# Autodesk Inventor assembly: 組合檔
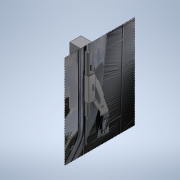
[picture p0: Inventor's stored thumbnail of the model, 180x180]
Saved by Autodesk Inventor 2020 (Build 240168000, 168)
## iProperties
Created: 2015-11-28
Part Number: 組合檔
Document SubType Name: Assembly
Designer: 設計製圖
Author: 設計製圖
## Documents named in this file (14)
- D:\資料庫\設計-3D Project\【May club 】\得利卡-車頂燈架\模型、圖面\22.01.05_設變 (未生產 )\短-車頂燈架-組合(#11.02)-總組合.iam
- D:\資料庫\設計-3D Project\材料庫\【螺絲】\止付螺絲\止付螺絲-M8-20.ipt
- D:\資料庫\設計-3D Project\【May club 】\得利卡-車頂燈架\模型、圖面\車身圖.ipt
- D:\資料庫\設計-3D Project\【May club 】\得利卡-車頂燈架\模型、圖面\得利卡-車頂導水槽.ipt
- D:\資料庫\設計-3D Project\材料庫\【螺絲】\外六角螺絲\白鐵-外六角  M6-20.ipt
- D:\資料庫\設計-3D Project\材料庫\【華司】\白鐵-平面華司-7-16-2t.ipt
- D:\資料庫\設計-3D Project\材料庫\【華司】\彈簧華司\白鐵-彈簧華司-6.ipt
- D:\資料庫\設計-3D Project\【May club 】\得利卡-車頂燈架\模型、圖面\短-車頂燈架-組合(#11.02)-生產圖面_21.11.26\製程筆記\封邊條 ( 平光黑 ) - 130L.ipt
- D:\資料庫\設計-3D Project\【May club 】\得利卡-車頂燈架\模型、圖面\短-車頂燈架-組合(#11.02)-生產圖面_21.11.26\製程筆記\背膠海綿eva 6T -  15W x 125L.ipt
- D:\資料庫\設計-3D Project\【May club 】\得利卡-車頂燈架\模型、圖面\短-車頂燈架-組合(#11.02)-生產圖面_21.11.26\製程筆記\背膠海綿eva 3T -  25W x 125L.ipt
- D:\資料庫\設計-3D Project\【May club 】\得利卡-車頂燈架\模型、圖面\短-車頂燈架-組合(#11.02)-生產圖面_21.11.26\製程筆記\背膠海綿eva 3T -  10W x 125L.ipt
- D:\資料庫\設計-3D Project\【May club 】\得利卡-車頂燈架\模型、圖面\22.01.05_設變 (未生產 )\吊架-短(R)(#01.05) - 焊接組合.iam
- D:\資料庫\設計-3D Project\【May club 】\得利卡-車頂燈架\模型、圖面\22.01.05_設變 (未生產 )\ㄇ槽(#01.05)- 焊接組合.iam
- D:\資料庫\設計-3D Project\【 鐵蹄 】\------鐵蹄工廠素材------ -\拉帽-M8.ipt
## Components (15 placed, 13 different names)
1. 吊架-短(R)(#01.05) - 焊接組合:1 [sub-assembly] — 貼合:68, 貼合:69, 齊平:13, 貼合:70, 貼合:74, 貼合:75, 齊平:15, 貼合:79, 貼合:80, 齊平:17, 貼合:81, 角度:1
2. ㄇ槽(#01.05)- 焊接組合:1 [sub-assembly] — 貼合:63, 貼合:64, 貼合:65, 貼合:66, 貼合:70, 貼合:71, 貼合:72, 貼合:73, 齊平:14, 貼合:76, 齊平:16, 齊平:17, 貼合:81, 角度:2
3. 拉帽-M8:1 — 貼合:63, 貼合:64, 貼合:67, 貼合:78
4. 拉帽-M8:2 — 貼合:65, 貼合:66, 貼合:67, 貼合:77
5. 得利卡-車頂導水槽:1
6. 車身圖:1
7. 背膠海綿eva 6T -  15W x 125L:1 — 貼合:74, 貼合:75, 齊平:15
8. 背膠海綿eva 3T -  25W x 125L:1 — 貼合:62, 貼合:72, 貼合:73, 齊平:14
9. 背膠海綿eva 3T -  10W x 125L:1 — 貼合:62, 貼合:76, 齊平:16
10. 白鐵-彈簧華司-6:1 — 貼合:49, 貼合:51, 貼合:52
11. 白鐵-平面華司-7-16-2t:1 — 貼合:48, 貼合:51, 貼合:80
12. 白鐵-外六角  M6-20:1 — 貼合:48, 貼合:49, 貼合:52, 貼合:71
13. 封邊條 ( 平光黑 ) - 130L:1 — 貼合:68, 貼合:69, 齊平:13
14. 止付螺絲-M8-20:1 — 齊平:12, 貼合:78, 貼合:79
15. 止付螺絲-M8-20:2 — 齊平:12, 貼合:77
## Relationships (32: Mate 24, Flush 6, Angle 2)
- 齊平:12 [Flush]: 止付螺絲-M8-20:1 ↔ 止付螺絲-M8-20:2
- 貼合:48 [Mate]: 白鐵-平面華司-7-16-2t:1 ↔ 白鐵-外六角  M6-20:1
- 貼合:49 [Mate]: 白鐵-彈簧華司-6:1 ↔ 白鐵-外六角  M6-20:1
- 貼合:51 [Mate]: 白鐵-彈簧華司-6:1 ↔ 白鐵-平面華司-7-16-2t:1
- 貼合:52 [Mate]: 白鐵-彈簧華司-6:1 ↔ 白鐵-外六角  M6-20:1
- 貼合:62 [Mate]: 背膠海綿eva 3T -  25W x 125L:1 ↔ 背膠海綿eva 3T -  10W x 125L:1
- 貼合:63 [Mate]: ㄇ槽(#01.05)- 焊接組合:1 ↔ 拉帽-M8:1
- 貼合:64 [Mate]: ㄇ槽(#01.05)- 焊接組合:1 ↔ 拉帽-M8:1
- 貼合:65 [Mate]: ㄇ槽(#01.05)- 焊接組合:1 ↔ 拉帽-M8:2
- 貼合:66 [Mate]: ㄇ槽(#01.05)- 焊接組合:1 ↔ 拉帽-M8:2
- 貼合:67 [Mate]: 拉帽-M8:1 ↔ 拉帽-M8:2
- 貼合:68 [Mate]: 吊架-短(R)(#01.05) - 焊接組合:1 ↔ 封邊條 ( 平光黑 ) - 130L:1
- 貼合:69 [Mate]: 吊架-短(R)(#01.05) - 焊接組合:1 ↔ 封邊條 ( 平光黑 ) - 130L:1
- 齊平:13 [Flush]: 吊架-短(R)(#01.05) - 焊接組合:1 ↔ 封邊條 ( 平光黑 ) - 130L:1
- 貼合:70 [Mate]: 吊架-短(R)(#01.05) - 焊接組合:1 ↔ ㄇ槽(#01.05)- 焊接組合:1
- 貼合:71 [Mate]: ㄇ槽(#01.05)- 焊接組合:1 ↔ 白鐵-外六角  M6-20:1
- 貼合:72 [Mate]: ㄇ槽(#01.05)- 焊接組合:1 ↔ 背膠海綿eva 3T -  25W x 125L:1
- 貼合:73 [Mate]: ㄇ槽(#01.05)- 焊接組合:1 ↔ 背膠海綿eva 3T -  25W x 125L:1
- 齊平:14 [Flush]: ㄇ槽(#01.05)- 焊接組合:1 ↔ 背膠海綿eva 3T -  25W x 125L:1
- 貼合:74 [Mate]: 吊架-短(R)(#01.05) - 焊接組合:1 ↔ 背膠海綿eva 6T -  15W x 125L:1
- 貼合:75 [Mate]: 吊架-短(R)(#01.05) - 焊接組合:1 ↔ 背膠海綿eva 6T -  15W x 125L:1
- 齊平:15 [Flush] (2 mm): 吊架-短(R)(#01.05) - 焊接組合:1 ↔ 背膠海綿eva 6T -  15W x 125L:1
- 貼合:76 [Mate]: ㄇ槽(#01.05)- 焊接組合:1 ↔ 背膠海綿eva 3T -  10W x 125L:1
- 齊平:16 [Flush]: ㄇ槽(#01.05)- 焊接組合:1 ↔ 背膠海綿eva 3T -  10W x 125L:1
- 貼合:77 [Mate]: 拉帽-M8:2 ↔ 止付螺絲-M8-20:2
- 貼合:78 [Mate]: 拉帽-M8:1 ↔ 止付螺絲-M8-20:1
- 貼合:79 [Mate]: 吊架-短(R)(#01.05) - 焊接組合:1 ↔ 止付螺絲-M8-20:1
- 貼合:80 [Mate]: 吊架-短(R)(#01.05) - 焊接組合:1 ↔ 白鐵-平面華司-7-16-2t:1
- 齊平:17 [Flush]: 吊架-短(R)(#01.05) - 焊接組合:1 ↔ ㄇ槽(#01.05)- 焊接組合:1
- 貼合:81 [Mate]: 吊架-短(R)(#01.05) - 焊接組合:1 ↔ ㄇ槽(#01.05)- 焊接組合:1
- 角度:1 [Angle] (180 deg): 吊架-短(R)(#01.05) - 焊接組合:1
- 角度:2 [Angle] (0 deg): ㄇ槽(#01.05)- 焊接組合:1
